# Autodesk Inventor assembly: jigForHexBushing
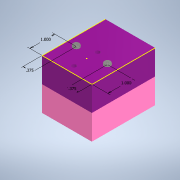
[picture p0: Inventor's stored thumbnail of the model, 180x180]
Saved by Autodesk Inventor 2022.1 (Build 261234000, 234)
## iProperties
Created: 2021-07-26
Part Number: jigForHexBushing
Document SubType Name: Assembly
Designer: robst
Author: robst
## Documents named in this file (4)
- C:\git\CAD-Development\robSteele\ShapeWays\TelescopeProjects\TelescopeMountNov2020\jigForHexBushing.iam
- C:\git\CAD-Development\robSteele\ShapeWays\TelescopeProjects\TelescopeMountNov2020\jigForHexBushingForConnectorPieceBottom.ipt
- C:\git\CAD-Development\robSteele\ShapeWays\TelescopeProjects\TelescopeMountNov2020\jigForHexBushingForConnectorPieceTop.ipt
- C:\Users\robst\Documents\Inventor\Content Center Files\R2021\en-US\ANSI B18.3(11)\ANSI B18.3 - 6-32 UNC - 2.25(23).ipt
## Components (4 placed, 3 different names)
1. jigForHexBushingForConnectorPieceBottom:1 — Mate:1, Flush:1, Flush:2
2. jigForHexBushingForConnectorPieceTop:1 — Mate:1, Flush:1, Flush:2, Mate:2, Mate:3, Mate:4, Mate:5
3. Spline Socket Button Head Cap Screw - Inch 6-32 UNC - 2.25:1 — Mate:2, Mate:3
4. Spline Socket Button Head Cap Screw - Inch 6-32 UNC - 2.25:2 — Mate:4, Mate:5
## Relationships (7: Mate 5, Flush 2)
- Mate:1: jigForHexBushingForConnectorPieceBottom:1 ↔ jigForHexBushingForConnectorPieceTop:1
- Flush:1: jigForHexBushingForConnectorPieceBottom:1 ↔ jigForHexBushingForConnectorPieceTop:1
- Flush:2: jigForHexBushingForConnectorPieceBottom:1 ↔ jigForHexBushingForConnectorPieceTop:1
- Mate:2: jigForHexBushingForConnectorPieceTop:1 ↔ Spline Socket Button Head Cap Screw - Inch 6-32 UNC - 2.25:1
- Mate:3: jigForHexBushingForConnectorPieceTop:1 ↔ Spline Socket Button Head Cap Screw - Inch 6-32 UNC - 2.25:1
- Mate:4: jigForHexBushingForConnectorPieceTop:1 ↔ Spline Socket Button Head Cap Screw - Inch 6-32 UNC - 2.25:2
- Mate:5: jigForHexBushingForConnectorPieceTop:1 ↔ Spline Socket Button Head Cap Screw - Inch 6-32 UNC - 2.25:2
